# Autodesk Inventor assembly: sprocket and bevel gear on shaft
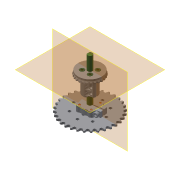
[picture p0: Inventor's stored thumbnail of the model, 180x180]
Saved by Autodesk Inventor 2019 (Build 230136000, 136)
## iProperties
Created: 2019-09-29
Part Number: sprocket and bevel gear on shaft
Document SubType Name: Assembly
Designer: ball
Author: ball
## Documents named in this file (4)
- C:\FTC\FTC8863CAD\2019 Robot\Mecanum Drive Train\sprocket and bevel gear on shaft.iam
- C:\FTC\FTC8863CAD\2019 Robot\Mecanum Drive Train\bevel gear with clamping hub.iam
- C:\FTC\FTC8863CAD\2019 Robot\Mecanum Drive Train\32 spocket with hub.iam
- C:\FTC\FTC8863CAD\2019 Robot\Mecanum Drive Train\3_2 shaft.ipt
## Components (3 placed, 3 different names)
1. 3_2 shaft:1
2. bevel gear with clamping hub:1 [sub-assembly] — Flush:2, Mate:8
3. 32 spocket with hub:1 [sub-assembly] — Mate:8
## Relationships (7: Mate 5, Angle 1, Flush 1)
- [Mate]: 3_2 shaft:1 ↔ 32 spocket with hub:1
- [Mate]: 3_2 shaft:1 ↔ bevel gear with clamping hub:1
- [Mate]: 3_2 shaft:1 ↔ bevel gear with clamping hub:1
- [Mate]: 3_2 shaft:1
- [Angle] (90 deg): 3_2 shaft:1
- Flush:2: bevel gear with clamping hub:1
- Mate:8 (12.2174 mm): bevel gear with clamping hub:1 ↔ 32 spocket with hub:1
